# Autodesk Inventor assembly: holes_check_full_itr2
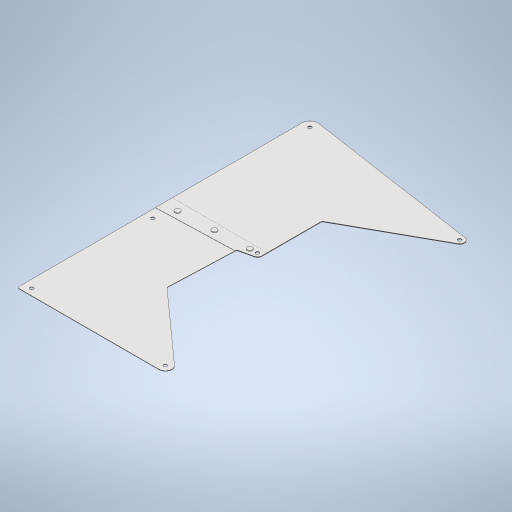
[picture p0: Inventor's stored thumbnail of the model, 512x512]
Saved by Autodesk Inventor 2024 (Build 280153000, 153)
## iProperties
Created: 2026-03-21
Part Number: holes_check_full_itr2
Document SubType Name: Assembly
Designer: schar
Author: schar
## Documents named in this file (4)
- C:\Users\schar\Desktop\tenSwitcHP\models\holes_check_full_itr2.iam
- C:\Users\schar\Desktop\tenSwitcHP\models\base_main_pcb_full_itr2.ipt
- C:\Users\schar\Desktop\tenSwitcHP\models\base_main_pcb_p1_itr2.ipt
- C:\Users\schar\Desktop\tenSwitcHP\models\base_main_pcb_p2_itr2.ipt
## Components (3 placed, 3 different names)
1. base_main_pcb_p1_itr2:1 — Mate:1, Mate:2, Mate:3, Mate:4, Flush:1
2. base_main_pcb_p2_itr2:1 — Mate:1, Mate:2, Mate:3, Flush:2
3. base_main_pcb_full_itr2:1 — Mate:4, Flush:1, Flush:2
## Relationships (6: Mate 4, Flush 2)
- Mate:1: base_main_pcb_p1_itr2:1 ↔ base_main_pcb_p2_itr2:1
- Mate:2: base_main_pcb_p1_itr2:1 ↔ base_main_pcb_p2_itr2:1
- Mate:3: base_main_pcb_p1_itr2:1 ↔ base_main_pcb_p2_itr2:1
- Mate:4: base_main_pcb_p1_itr2:1 ↔ base_main_pcb_full_itr2:1
- Flush:1: base_main_pcb_p1_itr2:1 ↔ base_main_pcb_full_itr2:1
- Flush:2: base_main_pcb_p2_itr2:1 ↔ base_main_pcb_full_itr2:1
